# Autodesk Inventor assembly: caterpillar_module_final_A
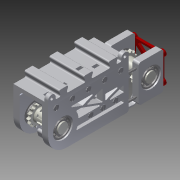
[picture p0: Inventor's stored thumbnail of the model, 180x180]
Saved by Autodesk Inventor 2015 (Build 190159000, 159)
## iProperties
Created: 2016-07-10
Part Number: caterpillar_module_final_A
Document SubType Name: Assembly
Designer: JavierPC
Author: JavierPC
## Documents named in this file (17)
- D:\Mis Documentos\TFM\CAD\v2\assembly\caterpillar_module_final_A.iam
- D:\Mis Documentos\TFM\CAD\v2\parts\combined_base_caterpillar_narrow_A_2.ipt
- D:\Mis Documentos\TFM\CAD\v2\parts\support_caterpillar_lateral_v3.ipt
- C:\Users\JavierPC\Documents\Inventor\Content Center Files\R2015\es-ES\DIN BEARING(1)\DIN 625 SKF - SKF 618_8.ipt
- D:\Mis Documentos\TFM\CAD\v2\parts\sprocket_encoder_axis_left_2.ipt
- D:\Mis Documentos\TFM\CAD\v2\parts\dumper_base_v1_SOCKET.ipt
- D:\Mis Documentos\TFM\CAD\v2\parts\spring_axis.ipt
- D:\Mis Documentos\TFM\CAD\v2\parts\support_caterpillar_spring_v1.3.ipt
- D:\Mis Documentos\TFM\CAD\v2\parts\sprocket_back_axis_2.ipt
- D:\Mis Documentos\TFM\CAD\v2\parts\Alignment_narrow.ipt
- D:\Mis Documentos\TFM\CAD\v2\parts\spring_final.iam
- C:\Users\JavierPC\Documents\Inventor\Content Center Files\R2015\es-ES\ISO 4032(1)\ISO 4032 - M2DIN EN.ipt
- C:\Users\JavierPC\Documents\Inventor\Content Center Files\R2015\es-ES\ISO 2009(1)\ISO 2009 - M2 x 12DIN EN 10.ipt
- D:\Mis Documentos\TFM\CAD\v2\parts\dumper_v9_NS.ipt
- D:\Mis Documentos\TFM\CAD\v2\parts\chain_path.ipt
- D:\Mis Documentos\TFM\CAD\v2\parts\chain_shoe.iam
- D:\Mis Documentos\TFM\CAD\v2\parts\link_joint_v4_z15_Dr1.5.ipt
## Components (112 placed, 16 different names)
1. combined_base_caterpillar_narrow_A_2:1 — Coincidencia:1, Coincidencia:2, Coincidencia:3, Coincidencia:4, Coincidencia:5, Coincidencia:6, Coincidencia:7, Nivelación:1, Coincidencia:11, Insertar:5, Insertar:6, Coincidencia:22, Coincidencia:26, Insertar:9, Ángulo:1, Insertar:10, Ángulo:2, Insertar:11, Ángulo:3, Insertar:12, Ángulo:4, Insertar:13, Ángulo:5, Insertar:28, Insertar:29, Insertar:30
2. support_caterpillar_lateral_v3:1 — Coincidencia:4, Coincidencia:5, Coincidencia:6, Coincidencia:8, Nivelación:2, Insertar:1, Insertar:2, Insertar:3, Insertar:4, Coincidencia:24, Insertar:20, Insertar:21, Insertar:22, Insertar:23, Insertar:24, Insertar:25, Insertar:26, Insertar:27, Coincidencia:105, Nivelación:102
3. sprocket_encoder_axis_left_2:1 — Coincidencia:9, Coincidencia:10, planoCentral
4. sprocket_back_axis_2:1 — Coincidencia:18, Coincidencia:19, Coincidencia:20
5. dumper_base_v1_SOCKET:1 — Coincidencia:11, Insertar:1, Insertar:2, Insertar:14, Ángulo:6, Insertar:15, Ángulo:7, Insertar:16, Ángulo:8, Insertar:17, Ángulo:9, Insertar:18, Ángulo:10, Insertar:19, Ángulo:11, Coincidencia:33, Coincidencia:34, Nivelación:6
6. dumper_v9_NS:1 — Coincidencia:33, Coincidencia:34, Nivelación:6
7. spring_axis:1 — Insertar:3, Coincidencia:14, Insertar:7
8. spring_axis:2 — Insertar:4, Coincidencia:15, Insertar:8, Coincidencia:25
9. spring_axis:3 — Insertar:5, Coincidencia:13, Coincidencia:27
10. spring_axis:4 — Insertar:6, Coincidencia:12, Coincidencia:23
11. support_caterpillar_spring_v1.3:1 — Coincidencia:14, Coincidencia:15, Coincidencia:16, Nivelación:3, Coincidencia:29, Coincidencia:30
12. support_caterpillar_spring_v1.3:2 — Coincidencia:12, Coincidencia:13, Coincidencia:17, Nivelación:4, Coincidencia:31, Coincidencia:32
13. Alignment_narrow:1 — Insertar:7, Insertar:8
14. chain_path:1 — planoCentral, Nivelación:37, Coincidencia:37, Nivelación:38, Coincidencia:39, Nivelación:39, Nivelación:40, Nivelación:41, Nivelación:42, Nivelación:43, Nivelación:44, Nivelación:45, Nivelación:46, Nivelación:47, Nivelación:48, Nivelación:49, Nivelación:50, Nivelación:51, Nivelación:52, Nivelación:53, Nivelación:54, Nivelación:55, Nivelación:56, Nivelación:57, Nivelación:58, Nivelación:59, Nivelación:60, Nivelación:61, Nivelación:62, Nivelación:63, Nivelación:64, Nivelación:65, Nivelación:66, Nivelación:67, Nivelación:68, Nivelación:69, Nivelación:70, Nivelación:71, Nivelación:72, Nivelación:73, Nivelación:74, Nivelación:75, Nivelación:76, Nivelación:77, Nivelación:78, Nivelación:79, Nivelación:80, Nivelación:81, Nivelación:82, Nivelación:83, Nivelación:84, Nivelación:85, Nivelación:86, Nivelación:87, Nivelación:88, Nivelación:89, Nivelación:90, Nivelación:91, Nivelación:92, Nivelación:93, Nivelación:94, Nivelación:95, Nivelación:96, Nivelación:97, Nivelación:98, Nivelación:99, Nivelación:100, Nivelación:101, Nivelación:103
15. link_joint_v4_z15_Dr1.5:43 — Nivelación:103, Coincidencia:106, Coincidencia:107
16. DIN 625 SKF 618/8:1 — Coincidencia:16, Nivelación:3, Coincidencia:20
17. DIN 625 SKF 618/8:2 — Coincidencia:17, Nivelación:4, Coincidencia:18, Coincidencia:19
18. DIN 625 SKF 618/8:3 — Coincidencia:8, Nivelación:2
19. DIN 625 SKF 618/8:4 — Coincidencia:7, Nivelación:1, Coincidencia:9, Coincidencia:10
20. spring_final:1 [sub-assembly] — Coincidencia:29, Coincidencia:105, Nivelación:102
21. spring_final:2 [sub-assembly] — Coincidencia:22, Coincidencia:23, Coincidencia:31
22. spring_final:3 [sub-assembly] — Coincidencia:24, Coincidencia:25, Coincidencia:30
23. spring_final:4 [sub-assembly] — Coincidencia:26, Coincidencia:27, Coincidencia:32
24. DIN EN 24032 M2:1 — Insertar:17, Ángulo:9
25. DIN EN 24032 M2:3 — Insertar:18, Ángulo:10
26. DIN EN 24032 M2:4 — Insertar:16, Ángulo:8
27. DIN EN 24032 M2:5 — Insertar:12, Ángulo:4
28. DIN EN 24032 M2:6 — Insertar:13, Ángulo:5
29. DIN EN 24032 M2:10 — Insertar:19, Ángulo:11
30. DIN EN 24032 M2:11 — Insertar:15, Ángulo:7
31. DIN EN 24032 M2:12 — Insertar:14, Ángulo:6
32. DIN EN 24032 M2:13 — Insertar:11, Ángulo:3
33. DIN EN 24032 M2:14 — Insertar:10, Ángulo:2
34. DIN EN 24032 M2:15 — Insertar:9, Ángulo:1
35. DIN EN ISO 2009 M2 x 12:1 — Insertar:20
36. DIN EN ISO 2009 M2 x 12:2 — Insertar:21
37. DIN EN ISO 2009 M2 x 12:3 — Insertar:22
38. DIN EN ISO 2009 M2 x 12:4 — Insertar:23
39. DIN EN ISO 2009 M2 x 12:5 — Insertar:24
40. DIN EN ISO 2009 M2 x 12:6 — Insertar:25
41. DIN EN ISO 2009 M2 x 12:7 — Insertar:26
42. DIN EN ISO 2009 M2 x 12:8 — Insertar:27
43. DIN EN ISO 2009 M2 x 12:9 — Insertar:28
44. DIN EN ISO 2009 M2 x 12:10 — Insertar:29
45. DIN EN ISO 2009 M2 x 12:11 — Insertar:30
46. chain_shoe:39 [sub-assembly] — Nivelación:98, Coincidencia:106
47. link_joint_v4_z15_Dr1.5:41 — Nivelación:99
48. chain_shoe:40 [sub-assembly] — Nivelación:100, Coincidencia:104
49. link_joint_v4_z15_Dr1.5:42 — Nivelación:101, Coincidencia:103, Coincidencia:104
50. chain_shoe:33 [sub-assembly] — Nivelación:97, Coincidencia:103
51. link_joint_v4_z15_Dr1.5:35 — Nivelación:96
52. chain_shoe:34 [sub-assembly] — Nivelación:95
53. link_joint_v4_z15_Dr1.5:36 — Nivelación:94
54. chain_shoe:35 [sub-assembly] — Nivelación:93
55. link_joint_v4_z15_Dr1.5:37 — Nivelación:92
56. chain_shoe:36 [sub-assembly] — Nivelación:91
57. link_joint_v4_z15_Dr1.5:38 — Nivelación:90
58. chain_shoe:37 [sub-assembly] — Nivelación:89
59. link_joint_v4_z15_Dr1.5:39 — Nivelación:88
60. chain_shoe:38 [sub-assembly] — Nivelación:87
61. link_joint_v4_z15_Dr1.5:40 — Nivelación:86, Coincidencia:99
62. chain_shoe:20 [sub-assembly] — Nivelación:60, Coincidencia:86
63. link_joint_v4_z15_Dr1.5:22 — Nivelación:61
64. chain_shoe:21 [sub-assembly] — Nivelación:62
65. link_joint_v4_z15_Dr1.5:23 — Nivelación:63
66. chain_shoe:22 [sub-assembly] — Nivelación:64
67. link_joint_v4_z15_Dr1.5:24 — Nivelación:65
68. chain_shoe:23 [sub-assembly] — Nivelación:66
69. link_joint_v4_z15_Dr1.5:25 — Nivelación:67
70. chain_shoe:24 [sub-assembly] — Nivelación:68
71. link_joint_v4_z15_Dr1.5:26 — Nivelación:69
72. chain_shoe:25 [sub-assembly] — Nivelación:70
73. link_joint_v4_z15_Dr1.5:27 — Nivelación:71
74. chain_shoe:26 [sub-assembly] — Nivelación:72
75. link_joint_v4_z15_Dr1.5:28 — Nivelación:73
76. chain_shoe:27 [sub-assembly] — Nivelación:74
77. link_joint_v4_z15_Dr1.5:29 — Nivelación:75
78. chain_shoe:28 [sub-assembly] — Nivelación:76
79. chain_shoe:29 [sub-assembly] — Nivelación:77
80. chain_shoe:30 [sub-assembly] — Nivelación:78
81. chain_shoe:31 [sub-assembly] — Nivelación:79
82. chain_shoe:32 [sub-assembly] — Nivelación:80, Coincidencia:107
83. link_joint_v4_z15_Dr1.5:30 — Nivelación:81
84. link_joint_v4_z15_Dr1.5:31 — Nivelación:82
85. link_joint_v4_z15_Dr1.5:32 — Nivelación:83
86. link_joint_v4_z15_Dr1.5:33 — Nivelación:84
87. link_joint_v4_z15_Dr1.5:34 — Nivelación:85, Coincidencia:86, Coincidencia:87
88. link_joint_v4_z15_Dr1.5:17 — Coincidencia:60, Nivelación:58, Coincidencia:61
89. link_joint_v4_z15_Dr1.5:18 — Coincidencia:56, Nivelación:54, Coincidencia:57
90. link_joint_v4_z15_Dr1.5:19 — Coincidencia:58, Nivelación:56, Coincidencia:59
91. chain_shoe:9 [sub-assembly] — Nivelación:51, Coincidencia:53, Coincidencia:54
92. link_joint_v4_z15_Dr1.5:21 — Coincidencia:54, Nivelación:52, Coincidencia:55
93. chain_shoe:10 [sub-assembly] — Nivelación:53, Coincidencia:55, Coincidencia:56
94. chain_shoe:11 [sub-assembly] — Nivelación:55, Coincidencia:57, Coincidencia:58
95. chain_shoe:16 [sub-assembly] — Nivelación:57, Coincidencia:59, Coincidencia:60
96. chain_shoe:19 [sub-assembly] — Nivelación:59, Coincidencia:61, Coincidencia:87
97. chain_shoe:5 [sub-assembly] — Nivelación:43, Coincidencia:52
98. link_joint_v4_z15_Dr1.5:5 — Nivelación:44
99. chain_shoe:6 [sub-assembly] — Nivelación:45
100. link_joint_v4_z15_Dr1.5:6 — Nivelación:46
101. chain_shoe:7 [sub-assembly] — Nivelación:47
102. link_joint_v4_z15_Dr1.5:7 — Nivelación:48
103. chain_shoe:8 [sub-assembly] — Nivelación:49
104. link_joint_v4_z15_Dr1.5:8 — Nivelación:50, Coincidencia:53
105. chain_shoe:3 [sub-assembly] — Nivelación:39, Coincidencia:44
106. link_joint_v4_z15_Dr1.5:3 — Nivelación:41
107. chain_shoe:4 [sub-assembly] — Nivelación:40
108. link_joint_v4_z15_Dr1.5:4 — Nivelación:42, Coincidencia:52
109. link_joint_v4_z15_Dr1.5:2 — Coincidencia:39, Coincidencia:44
110. chain_shoe:2 [sub-assembly] — Nivelación:38, Coincidencia:40
111. link_joint_v4_z15_Dr1.5:1 — Coincidencia:36, Coincidencia:37, Coincidencia:40
112. chain_shoe:1 [sub-assembly] — Nivelación:37, Coincidencia:36, Coincidencia:99
## Relationships (217: Mate 104, Flush 72, Insert 30, Angle 11)
- Coincidencia:1 [Mate]: combined_base_caterpillar_narrow_A_2:1
- Coincidencia:2 [Mate]: combined_base_caterpillar_narrow_A_2:1
- Coincidencia:3 [Mate]: combined_base_caterpillar_narrow_A_2:1
- Coincidencia:4 [Mate]: combined_base_caterpillar_narrow_A_2:1 ↔ support_caterpillar_lateral_v3:1
- Coincidencia:5 [Mate]: combined_base_caterpillar_narrow_A_2:1 ↔ support_caterpillar_lateral_v3:1
- Coincidencia:6 [Mate]: combined_base_caterpillar_narrow_A_2:1 ↔ support_caterpillar_lateral_v3:1
- Coincidencia:7 [Mate]: combined_base_caterpillar_narrow_A_2:1 ↔ DIN 625 SKF 618/8:4
- Nivelación:1 [Flush]: combined_base_caterpillar_narrow_A_2:1 ↔ DIN 625 SKF 618/8:4
- Coincidencia:8 [Mate]: support_caterpillar_lateral_v3:1 ↔ DIN 625 SKF 618/8:3
- Nivelación:2 [Flush]: support_caterpillar_lateral_v3:1 ↔ DIN 625 SKF 618/8:3
- Coincidencia:9 [Mate]: sprocket_encoder_axis_left_2:1 ↔ DIN 625 SKF 618/8:4
- Coincidencia:10 [Mate]: sprocket_encoder_axis_left_2:1 ↔ DIN 625 SKF 618/8:4
- Coincidencia:11 [Mate]: combined_base_caterpillar_narrow_A_2:1 ↔ dumper_base_v1_SOCKET:1
- Insertar:1: support_caterpillar_lateral_v3:1 ↔ dumper_base_v1_SOCKET:1
- Insertar:2: support_caterpillar_lateral_v3:1 ↔ dumper_base_v1_SOCKET:1
- Insertar:3: support_caterpillar_lateral_v3:1 ↔ spring_axis:1
- Insertar:4: support_caterpillar_lateral_v3:1 ↔ spring_axis:2
- Insertar:5: combined_base_caterpillar_narrow_A_2:1 ↔ spring_axis:3
- Insertar:6: combined_base_caterpillar_narrow_A_2:1 ↔ spring_axis:4
- Coincidencia:12 [Mate]: spring_axis:4 ↔ support_caterpillar_spring_v1.3:2
- Coincidencia:13 [Mate]: spring_axis:3 ↔ support_caterpillar_spring_v1.3:2
- Coincidencia:14 [Mate]: spring_axis:1 ↔ support_caterpillar_spring_v1.3:1
- Coincidencia:15 [Mate]: spring_axis:2 ↔ support_caterpillar_spring_v1.3:1
- Coincidencia:16 [Mate]: support_caterpillar_spring_v1.3:1 ↔ DIN 625 SKF 618/8:1
- Nivelación:3 [Flush]: support_caterpillar_spring_v1.3:1 ↔ DIN 625 SKF 618/8:1
- Coincidencia:17 [Mate]: support_caterpillar_spring_v1.3:2 ↔ DIN 625 SKF 618/8:2
- Nivelación:4 [Flush]: support_caterpillar_spring_v1.3:2 ↔ DIN 625 SKF 618/8:2
- Coincidencia:18 [Mate]: sprocket_back_axis_2:1 ↔ DIN 625 SKF 618/8:2
- Coincidencia:19 [Mate]: sprocket_back_axis_2:1 ↔ DIN 625 SKF 618/8:2
- Coincidencia:20 [Mate]: sprocket_back_axis_2:1 ↔ DIN 625 SKF 618/8:1
- Insertar:7: spring_axis:1 ↔ Alignment_narrow:1
- Insertar:8: spring_axis:2 ↔ Alignment_narrow:1
- Coincidencia:22 [Mate]: combined_base_caterpillar_narrow_A_2:1 ↔ spring_final:2
- Coincidencia:23 [Mate]: spring_axis:4 ↔ spring_final:2
- Coincidencia:24 [Mate]: support_caterpillar_lateral_v3:1 ↔ spring_final:3
- Coincidencia:25 [Mate]: spring_axis:2 ↔ spring_final:3
- Coincidencia:26 [Mate]: combined_base_caterpillar_narrow_A_2:1 ↔ spring_final:4
- Coincidencia:27 [Mate]: spring_axis:3 ↔ spring_final:4
- Coincidencia:29 [Mate]: support_caterpillar_spring_v1.3:1 ↔ spring_final:1
- Coincidencia:30 [Mate]: support_caterpillar_spring_v1.3:1 ↔ spring_final:3
- Coincidencia:31 [Mate]: support_caterpillar_spring_v1.3:2 ↔ spring_final:2
- Coincidencia:32 [Mate]: support_caterpillar_spring_v1.3:2 ↔ spring_final:4
- Insertar:9: combined_base_caterpillar_narrow_A_2:1 ↔ DIN EN 24032 M2:15
- Ángulo:1 [Angle] (0 deg): combined_base_caterpillar_narrow_A_2:1 ↔ DIN EN 24032 M2:15
- Insertar:10: combined_base_caterpillar_narrow_A_2:1 ↔ DIN EN 24032 M2:14
- Ángulo:2 [Angle] (0 deg): combined_base_caterpillar_narrow_A_2:1 ↔ DIN EN 24032 M2:14
- Insertar:11: combined_base_caterpillar_narrow_A_2:1 ↔ DIN EN 24032 M2:13
- Ángulo:3 [Angle] (0 deg): combined_base_caterpillar_narrow_A_2:1 ↔ DIN EN 24032 M2:13
- Insertar:12: combined_base_caterpillar_narrow_A_2:1 ↔ DIN EN 24032 M2:5
- Ángulo:4 [Angle] (0 deg): combined_base_caterpillar_narrow_A_2:1 ↔ DIN EN 24032 M2:5
- Insertar:13: combined_base_caterpillar_narrow_A_2:1 ↔ DIN EN 24032 M2:6
- Ángulo:5 [Angle] (0 deg): combined_base_caterpillar_narrow_A_2:1 ↔ DIN EN 24032 M2:6
- Insertar:14: dumper_base_v1_SOCKET:1 ↔ DIN EN 24032 M2:12
- Ángulo:6 [Angle] (0 deg): dumper_base_v1_SOCKET:1 ↔ DIN EN 24032 M2:12
- Insertar:15: dumper_base_v1_SOCKET:1 ↔ DIN EN 24032 M2:11
- Ángulo:7 [Angle] (0 deg): dumper_base_v1_SOCKET:1 ↔ DIN EN 24032 M2:11
- Insertar:16: dumper_base_v1_SOCKET:1 ↔ DIN EN 24032 M2:4
- Ángulo:8 [Angle] (0 deg): dumper_base_v1_SOCKET:1 ↔ DIN EN 24032 M2:4
- Insertar:17: dumper_base_v1_SOCKET:1 ↔ DIN EN 24032 M2:1
- Ángulo:9 [Angle] (0 deg): dumper_base_v1_SOCKET:1 ↔ DIN EN 24032 M2:1
- Insertar:18: dumper_base_v1_SOCKET:1 ↔ DIN EN 24032 M2:3
- Ángulo:10 [Angle] (0 deg): dumper_base_v1_SOCKET:1 ↔ DIN EN 24032 M2:3
- Insertar:19: dumper_base_v1_SOCKET:1 ↔ DIN EN 24032 M2:10
- Ángulo:11 [Angle] (0 deg): dumper_base_v1_SOCKET:1 ↔ DIN EN 24032 M2:10
- Insertar:20: support_caterpillar_lateral_v3:1 ↔ DIN EN ISO 2009 M2 x 12:1
- Insertar:21: support_caterpillar_lateral_v3:1 ↔ DIN EN ISO 2009 M2 x 12:2
- Insertar:22: support_caterpillar_lateral_v3:1 ↔ DIN EN ISO 2009 M2 x 12:3
- Insertar:23: support_caterpillar_lateral_v3:1 ↔ DIN EN ISO 2009 M2 x 12:4
- Insertar:24: support_caterpillar_lateral_v3:1 ↔ DIN EN ISO 2009 M2 x 12:5
- Insertar:25: support_caterpillar_lateral_v3:1 ↔ DIN EN ISO 2009 M2 x 12:6
- Insertar:26: support_caterpillar_lateral_v3:1 ↔ DIN EN ISO 2009 M2 x 12:7
- Insertar:27: support_caterpillar_lateral_v3:1 ↔ DIN EN ISO 2009 M2 x 12:8
- Insertar:28: combined_base_caterpillar_narrow_A_2:1 ↔ DIN EN ISO 2009 M2 x 12:9
- Insertar:29: combined_base_caterpillar_narrow_A_2:1 ↔ DIN EN ISO 2009 M2 x 12:10
- Insertar:30: combined_base_caterpillar_narrow_A_2:1 ↔ DIN EN ISO 2009 M2 x 12:11
- Coincidencia:33 [Mate]: dumper_base_v1_SOCKET:1 ↔ dumper_v9_NS:1
- Coincidencia:34 [Mate]: dumper_base_v1_SOCKET:1 ↔ dumper_v9_NS:1
- Nivelación:6 [Flush]: dumper_base_v1_SOCKET:1 ↔ dumper_v9_NS:1
- planoCentral [Mate]: sprocket_encoder_axis_left_2:1 ↔ chain_path:1
- Nivelación:37 [Flush]: chain_path:1 ↔ chain_shoe:1
- Coincidencia:36 [Mate]: link_joint_v4_z15_Dr1.5:1 ↔ chain_shoe:1
- Coincidencia:37 [Mate]: chain_path:1 ↔ link_joint_v4_z15_Dr1.5:1
- [Mate]: link_joint_v4_z15_Dr1.5:2 ↔ chain_shoe:2
- Nivelación:38 [Flush]: chain_path:1 ↔ chain_shoe:2
- Coincidencia:39 [Mate]: chain_path:1 ↔ link_joint_v4_z15_Dr1.5:2
- Coincidencia:40 [Mate]: chain_shoe:2 ↔ link_joint_v4_z15_Dr1.5:1
- [Mate]: chain_shoe:3 ↔ link_joint_v4_z15_Dr1.5:3
- [Mate]: chain_shoe:4 ↔ link_joint_v4_z15_Dr1.5:4
- [Mate]: link_joint_v4_z15_Dr1.5:3 ↔ chain_shoe:4
- Nivelación:39 [Flush]: chain_path:1 ↔ chain_shoe:3
- Nivelación:40 [Flush]: chain_path:1 ↔ chain_shoe:4
- Nivelación:41 [Flush]: chain_path:1 ↔ link_joint_v4_z15_Dr1.5:3
- Nivelación:42 [Flush]: chain_path:1 ↔ link_joint_v4_z15_Dr1.5:4
- Coincidencia:44 [Mate]: chain_shoe:3 ↔ link_joint_v4_z15_Dr1.5:2
- [Mate]: chain_shoe:5 ↔ link_joint_v4_z15_Dr1.5:5
- [Mate]: chain_shoe:6 ↔ link_joint_v4_z15_Dr1.5:6
- [Mate]: link_joint_v4_z15_Dr1.5:5 ↔ chain_shoe:6
- [Mate]: chain_shoe:7 ↔ link_joint_v4_z15_Dr1.5:7
- [Mate]: chain_shoe:8 ↔ link_joint_v4_z15_Dr1.5:8
- [Mate]: link_joint_v4_z15_Dr1.5:7 ↔ chain_shoe:8
- [Mate]: link_joint_v4_z15_Dr1.5:6 ↔ chain_shoe:7
- Nivelación:43 [Flush]: chain_path:1 ↔ chain_shoe:5
- Nivelación:44 [Flush]: chain_path:1 ↔ link_joint_v4_z15_Dr1.5:5
- Nivelación:45 [Flush]: chain_path:1 ↔ chain_shoe:6
- Nivelación:46 [Flush]: chain_path:1 ↔ link_joint_v4_z15_Dr1.5:6
- Nivelación:47 [Flush]: chain_path:1 ↔ chain_shoe:7
- Nivelación:48 [Flush]: chain_path:1 ↔ link_joint_v4_z15_Dr1.5:7
- Nivelación:49 [Flush]: chain_path:1 ↔ chain_shoe:8
- Nivelación:50 [Flush]: chain_path:1 ↔ link_joint_v4_z15_Dr1.5:8
- Coincidencia:52 [Mate]: chain_shoe:5 ↔ link_joint_v4_z15_Dr1.5:4
- Nivelación:51 [Flush]: chain_path:1 ↔ chain_shoe:9
- Coincidencia:53 [Mate]: chain_shoe:9 ↔ link_joint_v4_z15_Dr1.5:8
- Coincidencia:54 [Mate]: chain_shoe:9 ↔ link_joint_v4_z15_Dr1.5:21
- Nivelación:52 [Flush]: chain_path:1 ↔ link_joint_v4_z15_Dr1.5:21
- Nivelación:53 [Flush]: chain_path:1 ↔ chain_shoe:10
- Coincidencia:55 [Mate]: link_joint_v4_z15_Dr1.5:21 ↔ chain_shoe:10
- Coincidencia:56 [Mate]: link_joint_v4_z15_Dr1.5:18 ↔ chain_shoe:10
- Nivelación:54 [Flush]: chain_path:1 ↔ link_joint_v4_z15_Dr1.5:18
- Nivelación:55 [Flush]: chain_path:1 ↔ chain_shoe:11
- Coincidencia:57 [Mate]: link_joint_v4_z15_Dr1.5:18 ↔ chain_shoe:11
- Coincidencia:58 [Mate]: link_joint_v4_z15_Dr1.5:19 ↔ chain_shoe:11
- Nivelación:56 [Flush]: chain_path:1 ↔ link_joint_v4_z15_Dr1.5:19
- Nivelación:57 [Flush]: chain_path:1 ↔ chain_shoe:16
- Coincidencia:59 [Mate]: link_joint_v4_z15_Dr1.5:19 ↔ chain_shoe:16
- Coincidencia:60 [Mate]: link_joint_v4_z15_Dr1.5:17 ↔ chain_shoe:16
- Nivelación:58 [Flush]: chain_path:1 ↔ link_joint_v4_z15_Dr1.5:17
- Nivelación:59 [Flush]: chain_path:1 ↔ chain_shoe:19
- Coincidencia:61 [Mate]: link_joint_v4_z15_Dr1.5:17 ↔ chain_shoe:19
- [Mate]: chain_shoe:20 ↔ link_joint_v4_z15_Dr1.5:22
- [Mate]: chain_shoe:21 ↔ link_joint_v4_z15_Dr1.5:23
- [Mate]: link_joint_v4_z15_Dr1.5:22 ↔ chain_shoe:21
- [Mate]: chain_shoe:22 ↔ link_joint_v4_z15_Dr1.5:24
- [Mate]: chain_shoe:23 ↔ link_joint_v4_z15_Dr1.5:25
- [Mate]: link_joint_v4_z15_Dr1.5:24 ↔ chain_shoe:23
- [Mate]: link_joint_v4_z15_Dr1.5:23 ↔ chain_shoe:22
- [Mate]: chain_shoe:24 ↔ link_joint_v4_z15_Dr1.5:26
- [Mate]: chain_shoe:25 ↔ link_joint_v4_z15_Dr1.5:27
- [Mate]: link_joint_v4_z15_Dr1.5:26 ↔ chain_shoe:25
- [Mate]: chain_shoe:26 ↔ link_joint_v4_z15_Dr1.5:28
- [Mate]: chain_shoe:27 ↔ link_joint_v4_z15_Dr1.5:29
- [Mate]: link_joint_v4_z15_Dr1.5:28 ↔ chain_shoe:27
- [Mate]: link_joint_v4_z15_Dr1.5:27 ↔ chain_shoe:26
- [Mate]: link_joint_v4_z15_Dr1.5:25 ↔ chain_shoe:24
- [Mate]: link_joint_v4_z15_Dr1.5:29 ↔ chain_shoe:28
- [Mate]: chain_shoe:28 ↔ link_joint_v4_z15_Dr1.5:33
- [Mate]: chain_shoe:29 ↔ link_joint_v4_z15_Dr1.5:33
- [Mate]: chain_shoe:29 ↔ link_joint_v4_z15_Dr1.5:31
- [Mate]: chain_shoe:30 ↔ link_joint_v4_z15_Dr1.5:31
- [Mate]: chain_shoe:30 ↔ link_joint_v4_z15_Dr1.5:32
- [Mate]: chain_shoe:31 ↔ link_joint_v4_z15_Dr1.5:32
- [Mate]: chain_shoe:31 ↔ link_joint_v4_z15_Dr1.5:30
- [Mate]: chain_shoe:32 ↔ link_joint_v4_z15_Dr1.5:30
- Nivelación:60 [Flush]: chain_path:1 ↔ chain_shoe:20
- Nivelación:61 [Flush]: chain_path:1 ↔ link_joint_v4_z15_Dr1.5:22
- Nivelación:62 [Flush]: chain_path:1 ↔ chain_shoe:21
- Nivelación:63 [Flush]: chain_path:1 ↔ link_joint_v4_z15_Dr1.5:23
- Nivelación:64 [Flush]: chain_path:1 ↔ chain_shoe:22
- Nivelación:65 [Flush]: chain_path:1 ↔ link_joint_v4_z15_Dr1.5:24
- Nivelación:66 [Flush]: chain_path:1 ↔ chain_shoe:23
- Nivelación:67 [Flush]: chain_path:1 ↔ link_joint_v4_z15_Dr1.5:25
- Nivelación:68 [Flush]: chain_path:1 ↔ chain_shoe:24
- Nivelación:69 [Flush]: chain_path:1 ↔ link_joint_v4_z15_Dr1.5:26
- Nivelación:70 [Flush]: chain_path:1 ↔ chain_shoe:25
- Nivelación:71 [Flush]: chain_path:1 ↔ link_joint_v4_z15_Dr1.5:27
- Nivelación:72 [Flush]: chain_path:1 ↔ chain_shoe:26
- Nivelación:73 [Flush]: chain_path:1 ↔ link_joint_v4_z15_Dr1.5:28
- Nivelación:74 [Flush]: chain_path:1 ↔ chain_shoe:27
- Nivelación:75 [Flush]: chain_path:1 ↔ link_joint_v4_z15_Dr1.5:29
- Nivelación:76 [Flush]: chain_path:1 ↔ chain_shoe:28
- Nivelación:77 [Flush]: chain_path:1 ↔ chain_shoe:29
- Nivelación:78 [Flush]: chain_path:1 ↔ chain_shoe:30
- Nivelación:79 [Flush]: chain_path:1 ↔ chain_shoe:31
- Nivelación:80 [Flush]: chain_path:1 ↔ chain_shoe:32
- Nivelación:81 [Flush]: chain_path:1 ↔ link_joint_v4_z15_Dr1.5:30
- Nivelación:82 [Flush]: chain_path:1 ↔ link_joint_v4_z15_Dr1.5:31
- Nivelación:83 [Flush]: chain_path:1 ↔ link_joint_v4_z15_Dr1.5:32
- Nivelación:84 [Flush]: chain_path:1 ↔ link_joint_v4_z15_Dr1.5:33
- Nivelación:85 [Flush]: chain_path:1 ↔ link_joint_v4_z15_Dr1.5:34
- Coincidencia:86 [Mate]: chain_shoe:20 ↔ link_joint_v4_z15_Dr1.5:34
- Coincidencia:87 [Mate]: link_joint_v4_z15_Dr1.5:34 ↔ chain_shoe:19
- [Mate]: chain_shoe:33 ↔ link_joint_v4_z15_Dr1.5:35
- [Mate]: chain_shoe:34 ↔ link_joint_v4_z15_Dr1.5:36
- [Mate]: link_joint_v4_z15_Dr1.5:35 ↔ chain_shoe:34
- [Mate]: chain_shoe:35 ↔ link_joint_v4_z15_Dr1.5:37
- [Mate]: chain_shoe:36 ↔ link_joint_v4_z15_Dr1.5:38
- [Mate]: link_joint_v4_z15_Dr1.5:37 ↔ chain_shoe:36
- [Mate]: link_joint_v4_z15_Dr1.5:36 ↔ chain_shoe:35
- [Mate]: chain_shoe:37 ↔ link_joint_v4_z15_Dr1.5:39
- [Mate]: chain_shoe:38 ↔ link_joint_v4_z15_Dr1.5:40
- [Mate]: link_joint_v4_z15_Dr1.5:39 ↔ chain_shoe:38
- [Mate]: link_joint_v4_z15_Dr1.5:38 ↔ chain_shoe:37
- Nivelación:86 [Flush]: chain_path:1 ↔ link_joint_v4_z15_Dr1.5:40
- Nivelación:87 [Flush]: chain_path:1 ↔ chain_shoe:38
- Nivelación:88 [Flush]: chain_path:1 ↔ link_joint_v4_z15_Dr1.5:39
- Nivelación:89 [Flush]: chain_path:1 ↔ chain_shoe:37
- Nivelación:90 [Flush]: chain_path:1 ↔ link_joint_v4_z15_Dr1.5:38
- Nivelación:91 [Flush]: chain_path:1 ↔ chain_shoe:36
- Nivelación:92 [Flush]: chain_path:1 ↔ link_joint_v4_z15_Dr1.5:37
- Nivelación:93 [Flush]: chain_path:1 ↔ chain_shoe:35
- Nivelación:94 [Flush]: chain_path:1 ↔ link_joint_v4_z15_Dr1.5:36
- Nivelación:95 [Flush]: chain_path:1 ↔ chain_shoe:34
- Nivelación:96 [Flush]: chain_path:1 ↔ link_joint_v4_z15_Dr1.5:35
- Nivelación:97 [Flush]: chain_path:1 ↔ chain_shoe:33
- Coincidencia:99 [Mate]: link_joint_v4_z15_Dr1.5:40 ↔ chain_shoe:1
- [Mate]: chain_shoe:39 ↔ link_joint_v4_z15_Dr1.5:41
- [Mate]: link_joint_v4_z15_Dr1.5:41 ↔ chain_shoe:40
- Nivelación:98 [Flush]: chain_path:1 ↔ chain_shoe:39
- Nivelación:99 [Flush]: chain_path:1 ↔ link_joint_v4_z15_Dr1.5:41
- Nivelación:100 [Flush]: chain_path:1 ↔ chain_shoe:40
- Nivelación:101 [Flush]: chain_path:1 ↔ link_joint_v4_z15_Dr1.5:42
- Coincidencia:103 [Mate]: link_joint_v4_z15_Dr1.5:42 ↔ chain_shoe:33
- Coincidencia:104 [Mate]: chain_shoe:40 ↔ link_joint_v4_z15_Dr1.5:42
- Coincidencia:105 [Mate]: support_caterpillar_lateral_v3:1 ↔ spring_final:1
- Nivelación:102 [Flush]: support_caterpillar_lateral_v3:1 ↔ spring_final:1
- Nivelación:103 [Flush]: chain_path:1 ↔ link_joint_v4_z15_Dr1.5:43
- Coincidencia:106 [Mate]: link_joint_v4_z15_Dr1.5:43 ↔ chain_shoe:39
- Coincidencia:107 [Mate]: link_joint_v4_z15_Dr1.5:43 ↔ chain_shoe:32
## Named parameters: d87_d85 = 0 mm, d91_d90 = 0 mm, d92_d85 = 0 mm, d93_d87_d85 = 0 mm, d99_d90 = 0 mm, d100_d91_d90 = 0 mm, d101_d92_d85 = 0 mm, d102_d93_d87_d85 = 0 mm, d103_d98 = 0 mm, d104_d85 = 0 mm, d105_d87_d85 = 0 mm, d134_d125 = 0 mm, d135_d126 = 0 mm, d136_d129 = 0 mm, d137_d130 = 0 mm, d138_d133 = 0 mm, d139_d90 = 0 mm, d140_d91_d90 = 0 mm, d141_d92_d85 = 0 mm, d142_d93_d87_d85 = 0 mm, d143_d98 = 0 mm, d144_d99_d90 = 0 mm, d145_d100_d91_d90 = 0 mm, d146_d101_d92_d85 = 0 mm, d147_d102_d93_d87_d85 = 0 mm, d148_d103_d98 = 0 mm, d149_d104_d85 = 0 mm, d150_d105_d87_d85 = 0 mm, d151_d114 = 0 mm, d152_d116 = 0 mm, d153_d117 = 0 mm, d154_d120 = 0 mm, d155_d121 = 0 mm, d156_d85 = 0 mm, d157_d87_d85 = 0 mm, d186_d90 = 0 mm, d187_d91_d90 = 0 mm, d188_d92_d85 = 0 mm, d189_d93_d87_d85 = 0 mm, d190_d98 = 0 mm, d191_d99_d90 = 0 mm, d192_d104_d85 = 0 mm, d193_d105_d87_d85 = 0 mm, d194_d114 = 0 mm, d195_d85 = 0 mm, d196_d87_d85 = 0 mm, d210_d186_d90 = 0 mm, d211_d195_d85 = 0 mm
